# Autodesk Inventor assembly: frame
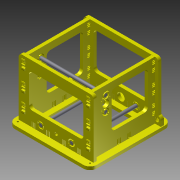
[picture p0: Inventor's stored thumbnail of the model, 180x180]
Saved by Autodesk Inventor 2012 SP1 (Build 160190100, 190)
## iProperties
Created: 2011-11-06
Part Number: frame
Document SubType Name: Assembly
Designer: Aaron
Author: Aaron
## Documents named in this file (8)
- C:\Users\Aaron\Documents\Projects\MTM-Snap-Metric\frame.iam
- C:\Users\Aaron\Documents\Projects\MTM-Snap-Metric\front.ipt
- C:\Users\Aaron\Documents\Projects\MTM-Snap-Metric\sideB.ipt
- C:\Users\Aaron\Documents\Projects\MTM-Snap-Metric\sideA.ipt
- C:\Users\Aaron\Documents\Projects\MTM-Snap-Metric\back.ipt
- C:\Users\Aaron\Documents\Projects\MTM-Snap-Metric\base.ipt
- C:\Users\Aaron\Documents\Projects\MTM-Snap-Metric\linear-guide-x.ipt
- C:\Users\Aaron\Documents\Projects\MTM-Snap-Metric\linear-guide-y.ipt
## Components (9 placed, 7 different names)
1. front:1 — Mate:1, Mate:2, Flush:1, Mate:3, Flush:2, Mate:4, Insert:1, Insert:2
2. sideB:1 — Mate:1, Mate:2, Flush:1, Mate:5, Insert:3, Insert:4
3. sideA:1 — Mate:3, Flush:2, Mate:4, Flush:3, Mate:6, Mate:7, Mate:9
4. back:1 — Flush:3, Mate:5, Mate:6, Mate:8
5. base:1 — Mate:7, Mate:8, Mate:9
6. linear-guide-x:1 — Insert:1
7. linear-guide-x:2 — Insert:2
8. linear-guide-y:1 — Insert:3
9. linear-guide-y:2 — Insert:4
## Relationships (16: Mate 9, Insert 4, Flush 3)
- Mate:1: front:1 ↔ sideB:1
- Mate:2: front:1 ↔ sideB:1
- Flush:1: front:1 ↔ sideB:1
- Mate:3: front:1 ↔ sideA:1
- Flush:2: front:1 ↔ sideA:1
- Mate:4: front:1 ↔ sideA:1
- Flush:3: sideA:1 ↔ back:1
- Mate:5: sideB:1 ↔ back:1
- Mate:6: sideA:1 ↔ back:1
- Mate:7: sideA:1 ↔ base:1
- Mate:8: back:1 ↔ base:1
- Mate:9: sideA:1 ↔ base:1
- Insert:1: front:1 ↔ linear-guide-x:1
- Insert:2: front:1 ↔ linear-guide-x:2
- Insert:3: sideB:1 ↔ linear-guide-y:1
- Insert:4: sideB:1 ↔ linear-guide-y:2
